# Autodesk Inventor assembly: axis3
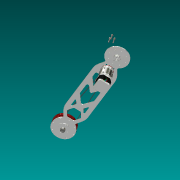
[picture p0: Inventor's stored thumbnail of the model, 180x180]
Saved by Autodesk Inventor 2020.3 (Build 243373000, 373)
## iProperties
Created: 2020-05-24
Part Number: axis3
Document SubType Name: Assembly
Designer: Svend
Author: Svend
## Documents named in this file (14)
- C:\Users\Svend\OneDrive\Documents\GitHub\BeerMinder\3D-model\axis3\axis3.iam
- C:\Users\Svend\OneDrive\Documents\GitHub\BeerMinder\3D-model\subAssembly\Nema17MetGearbox.iam
- C:\Users\Svend\OneDrive\Documents\GitHub\BeerMinder\3D-model\pulleys\GT2 Timing Pulley 20T - 8mm as.ipt
- C:\Users\Svend\OneDrive\Documents\GitHub\BeerMinder\3D-model\pulleys\Tandriem20naar60T-696mm.ipt
- C:\Users\Svend\OneDrive\Documents\GitHub\BeerMinder\3D-model\Base (Axis 1)\spiebaanBevestiging.ipt
- C:\Users\Svend\OneDrive\Documents\GitHub\BeerMinder\3D-model\pulleys\GT2 Timing Pulley 60T - 8mm as.ipt
- C:\Users\Svend\OneDrive\Documents\GitHub\BeerMinder\3D-model\bearings\Ball Bearing 608ZZ.ipt
- C:\Users\Svend\OneDrive\Documents\GitHub\BeerMinder\3D-model\Base (Axis 1)\asArm2.ipt
- C:\Users\Svend\OneDrive\Documents\GitHub\BeerMinder\3D-model\Base (Axis 1)\arm1v2.ipt
- C:\Users\Svend\OneDrive\Documents\GitHub\BeerMinder\3D-model\Base (Axis 1)\60mmspacer.ipt
- C:\Users\Svend\OneDrive\Documents\GitHub\BeerMinder\3D-model\Base (Axis 1)\60mmspacerDicht.ipt
- C:\Users\Svend\OneDrive\Documents\GitHub\BeerMinder\3D-model\bearings\stelring - 8mm.ipt
- C:\Users\Svend\OneDrive\Documents\Inventor\Content Center Files\R2020\en-US\ISO 4762(2)\ISO 4762 - M4 x 20ISO.ipt
- C:\Users\Svend\OneDrive\Documents\GitHub\BeerMinder\3D-model\axis4\spacerVoorLager.ipt
## Components (15 placed, 13 different names)
1. Nema17MetGearbox:1 [sub-assembly]
2. GT2 Timing Pulley 20T - 8mm as:1
3. Tandriem20naar60T-696mm:1
4. spiebaanBevestiging:1
5. GT2 Timing Pulley 60T - 8mm as:1
6. Ball Bearing 608ZZ:1
7. asArm2:1
8. arm1v2:1 — Mate:22, Mate:23, Mate:24
9. 60mmspacer:1
10. 60mmspacerDicht:1
11. stelring - 8mm:1
12. ISO 4762 M4 x 20:1
13. ISO 4762 M4 x 20:2
14. ISO 4762 M4 x 20:3
15. spacerVoorLager:1 — Mate:22, Mate:23, Mate:24
## Relationships (28: Mate 24, Flush 3, Angle 1)
- [Mate]: GT2 Timing Pulley 20T - 8mm as:1 ↔ Tandriem20naar60T-696mm:1
- [Mate]: Tandriem20naar60T-696mm:1 ↔ GT2 Timing Pulley 60T - 8mm as:1
- [Mate] (0.5 mm): Tandriem20naar60T-696mm:1 ↔ GT2 Timing Pulley 60T - 8mm as:1
- [Mate]: GT2 Timing Pulley 60T - 8mm as:1 ↔ Ball Bearing 608ZZ:1
- [Mate]: GT2 Timing Pulley 60T - 8mm as:1 ↔ Ball Bearing 608ZZ:1
- [Mate]: Ball Bearing 608ZZ:1 ↔ asArm2:1
- [Mate]: spiebaanBevestiging:1 ↔ arm1v2:1
- [Flush]: spiebaanBevestiging:1 ↔ arm1v2:1
- [Mate]: Nema17MetGearbox:1 ↔ arm1v2:1
- [Angle] (180 deg): Nema17MetGearbox:1 ↔ arm1v2:1
- [Mate]: Nema17MetGearbox:1 ↔ GT2 Timing Pulley 20T - 8mm as:1
- [Mate] (0.5 mm): GT2 Timing Pulley 20T - 8mm as:1 ↔ Tandriem20naar60T-696mm:1
- [Mate]: Nema17MetGearbox:1 ↔ arm1v2:1
- [Mate]: arm1v2:1 ↔ 60mmspacer:1
- [Mate]: arm1v2:1 ↔ 60mmspacer:1
- [Mate]: arm1v2:1 ↔ 60mmspacer:1
- [Flush]: Ball Bearing 608ZZ:1 ↔ 60mmspacer:1
- [Mate]: 60mmspacer:1 ↔ 60mmspacerDicht:1
- [Mate]: 60mmspacer:1 ↔ 60mmspacerDicht:1
- [Mate]: 60mmspacer:1 ↔ 60mmspacerDicht:1
- [Mate]: asArm2:1 ↔ stelring - 8mm:1
- [Mate]: 60mmspacerDicht:1 ↔ stelring - 8mm:1
- [Flush]: asArm2:1 ↔ stelring - 8mm:1
- [Mate]: arm1v2:1 ↔ stelring - 8mm:1
- [Mate]: spiebaanBevestiging:1 ↔ arm1v2:1
- Mate:22: arm1v2:1 ↔ spacerVoorLager:1
- Mate:23: arm1v2:1 ↔ spacerVoorLager:1
- Mate:24: arm1v2:1 ↔ spacerVoorLager:1
